# Autodesk Inventor assembly: CHASSI
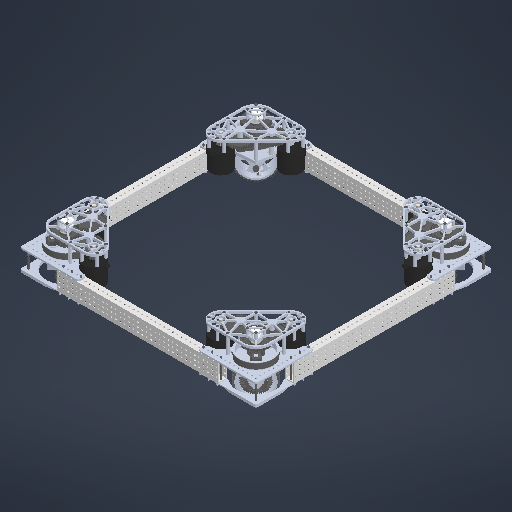
[picture p0: Inventor's stored thumbnail of the model, 512x512]
Saved by Autodesk Inventor 2026 (Build 300175000, 175)
## iProperties
Created: 2026-06-15
Part Number: CHASSI
Document SubType Name: Assembly
Designer: DELL
Author: DELL
## Documents named in this file (3)
- C:\Users\DELL\OneDrive - SFIEMT\Área de Trabalho\PROJETO FRC\CAD\CHASSI.iam
- C:\Users\DELL\OneDrive - SFIEMT\Área de Trabalho\PROJETO FRC\CAD\CHASSI\SWEERVE\MK4I NEO v1.iam
- C:\Users\DELL\OneDrive - SFIEMT\Área de Trabalho\PROJETO FRC\CAD\CHASSI\PERFIL 50X25 STEMOS 469MM.ipt
## Components (8 placed, 2 different names)
1. MK4I NEO v1:1 [sub-assembly] — Alinhado:1, Alinhado:2, Alinhado:6, Coincidente:1, Coincidente:3, Coincidente:4, Coincidente:14
2. MK4I NEO v1:2 [sub-assembly] — Alinhado:3, Alinhado:4, Alinhado:5, Alinhado:7, Coincidente:2, Coincidente:8, Coincidente:11
3. MK4I NEO v1:3 [sub-assembly] — Alinhado:5, Alinhado:6, Alinhado:7, Coincidente:5, Coincidente:6, Coincidente:7
4. MK4I NEO v1:4 [sub-assembly] — Alinhado:1, Alinhado:2, Alinhado:3, Alinhado:4, Coincidente:1, Coincidente:2, Coincidente:9, Coincidente:10, Coincidente:12, Coincidente:13
5. PERFIL 50X25 STEMOS 469MM:1 — Coincidente:3, Coincidente:4, Coincidente:5
6. PERFIL 50X25 STEMOS 469MM:2 — Coincidente:12, Coincidente:13, Coincidente:14
7. PERFIL 50X25 STEMOS 469MM:3 — Coincidente:9, Coincidente:10, Coincidente:11
8. PERFIL 50X25 STEMOS 469MM:4 — Coincidente:6, Coincidente:7, Coincidente:8
## Relationships (21: Mate 14, Flush 7)
- Alinhado:1 [Flush]: MK4I NEO v1:1 ↔ MK4I NEO v1:4
- Alinhado:2 [Flush]: MK4I NEO v1:1 ↔ MK4I NEO v1:4
- Alinhado:3 [Flush]: MK4I NEO v1:2 ↔ MK4I NEO v1:4
- Alinhado:4 [Flush]: MK4I NEO v1:2 ↔ MK4I NEO v1:4
- Alinhado:5 [Flush]: MK4I NEO v1:2 ↔ MK4I NEO v1:3
- Alinhado:6 [Flush]: MK4I NEO v1:1 ↔ MK4I NEO v1:3
- Alinhado:7 [Flush]: MK4I NEO v1:2 ↔ MK4I NEO v1:3
- Coincidente:1 [Mate] (-685.8 mm): MK4I NEO v1:1 ↔ MK4I NEO v1:4
- Coincidente:2 [Mate] (-685.8 mm): MK4I NEO v1:2 ↔ MK4I NEO v1:4
- Coincidente:3 [Mate]: MK4I NEO v1:1 ↔ PERFIL 50X25 STEMOS 469MM:1
- Coincidente:4 [Mate]: MK4I NEO v1:1 ↔ PERFIL 50X25 STEMOS 469MM:1
- Coincidente:5 [Mate]: MK4I NEO v1:3 ↔ PERFIL 50X25 STEMOS 469MM:1
- Coincidente:6 [Mate]: MK4I NEO v1:3 ↔ PERFIL 50X25 STEMOS 469MM:4
- Coincidente:7 [Mate]: MK4I NEO v1:3 ↔ PERFIL 50X25 STEMOS 469MM:4
- Coincidente:8 [Mate]: MK4I NEO v1:2 ↔ PERFIL 50X25 STEMOS 469MM:4
- Coincidente:9 [Mate]: MK4I NEO v1:4 ↔ PERFIL 50X25 STEMOS 469MM:3
- Coincidente:10 [Mate]: MK4I NEO v1:4 ↔ PERFIL 50X25 STEMOS 469MM:3
- Coincidente:11 [Mate]: MK4I NEO v1:2 ↔ PERFIL 50X25 STEMOS 469MM:3
- Coincidente:12 [Mate]: MK4I NEO v1:4 ↔ PERFIL 50X25 STEMOS 469MM:2
- Coincidente:13 [Mate]: MK4I NEO v1:4 ↔ PERFIL 50X25 STEMOS 469MM:2
- Coincidente:14 [Mate]: MK4I NEO v1:1 ↔ PERFIL 50X25 STEMOS 469MM:2
